# Autodesk Inventor assembly: 16631023
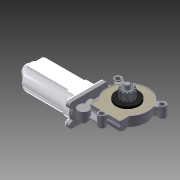
[picture p0: Inventor's stored thumbnail of the model, 180x180]
Saved by Autodesk Inventor 2011 (Build 150239000, 239)
## iProperties
Category: Motors
Created: 2007-12-06
Part Number: 16631023
Document SubType Name: Assembly
Project: FIRST
Description: Motor - Keyang LH 12 tooth pinion
Vendor: Keyang
Mass: 850 g
Surface Area: 430.457 cm^2
Volume: 226.7 cm^3
Title: Motor - Keyang LH 12 tooth pinion
Author: Autodesk, Inc.
## Documents named in this file (3)
- R:\2012\Inventor\vkop\All_Motors\Motors_Keyang_16631023.iam
- R:\2012\Inventor\vkop\All_Motors\16631023_body_LH.ipt
- R:\2012\Inventor\vkop\All_Motors\16631023_12 tooth pinion gear.ipt
## Components (2 placed, 2 different names)
1. 16631023_body_LH:1 — Mate:1
2. 16631023_12 tooth pinion gear:1 — Mate:1
## Relationships (2: Mate 2)
- Mate:1: 16631023_body_LH:1 ↔ 16631023_12 tooth pinion gear:1
- [Mate]: 16631023_body_LH:1 ↔ 16631023_12 tooth pinion gear:1
